# Autodesk Inventor assembly: Gripper Attempt 04
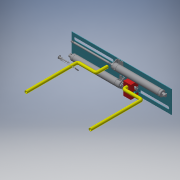
[picture p0: Inventor's stored thumbnail of the model, 180x180]
Saved by Autodesk Inventor 2016 (Build 200138000, 138)
## iProperties
Created: 2015-06-19
Part Number: Gripper Attempt 04
Document SubType Name: Assembly
Designer: steele
Mass: 1782.14 g
Surface Area: 5525.09 cm^2
Volume: 900.724 cm^3
Density: 1.97857 g/cm^3
Author: steele
## Documents named in this file (9)
- C:\snobotics\CAD-Development\robSteele\SnoBoticsSummer2015\Gripper\Gripper Attempt 04.iam
- C:\snobotics\CAD-MfgResources\McMaster-Carr\Air Cylinder\Pivot Mount Cylinders\Foot Bracket for 1_25 and 1_50 Bore\6498K340.ipt
- C:\snobotics\CAD-Development\robSteele\SnoBoticsSummer2015\Gripper\6498K681.ipt
- C:\snobotics\CAD-Development\robSteele\ipartComponents\Plate for Gripper.ipt
- C:\snobotics\CAD-Development\robSteele\ipartComponents\Plate for Gripper\Plate for Gripper 6 x 27 x 1_8.ipt
- C:\snobotics\CAD-Development\robSteele\SnoBoticsSummer2015\Gripper\Support For Arms.ipt
- C:\snobotics\CAD-Development\robSteele\SnoBoticsSummer2015\Gripper\Support Overlay on Gripper Side.ipt
- C:\snobotics\CAD-Development\robSteele\ipartComponents\ABS Arm.ipt
- C:\snobotics\CAD-MfgResources\McMaster-Carr\Quick Release Pin\94748A227.ipt
## Components (11 placed, 7 different names)
1. Plate for Gripper 6 x 27 x 1_8:1 — Mate:1, Flush:1, Flush:2, Mate:2, Flush:3, Flush:4, Mate:9
2. 6498K340:1 — Mate:2, Flush:3, Flush:4, Mate:7
3. 6498K340:2 — Mate:1, Flush:1, Flush:2, Mate:8
4. 6498K681:1 — Mate:7
5. 6498K681:2 — Mate:8, Insert:3
6. Support For Arms:1 — Mate:9, Insert:3, Mate:10, Flush:10, Flush:13, Mate:12
7. Support Overlay on Gripper Side:1 — Mate:10, Flush:10, Flush:13, Mate:12, Insert:4, Insert:5
8. ABS Arm:1 — Insert:4
9. ABS Arm:2
10. 94748A227:1 — Insert:5
11. 94748A227:2
## Relationships (16: Mate 7, Flush 6, Insert 3)
- Mate:1: Plate for Gripper 6 x 27 x 1_8:1 ↔ 6498K340:2
- Flush:1: Plate for Gripper 6 x 27 x 1_8:1 ↔ 6498K340:2
- Flush:2 (330.2 mm): Plate for Gripper 6 x 27 x 1_8:1 ↔ 6498K340:2
- Mate:2: Plate for Gripper 6 x 27 x 1_8:1 ↔ 6498K340:1
- Flush:3: Plate for Gripper 6 x 27 x 1_8:1 ↔ 6498K340:1
- Flush:4 (330.2 mm): Plate for Gripper 6 x 27 x 1_8:1 ↔ 6498K340:1
- Mate:7: 6498K340:1 ↔ 6498K681:1
- Mate:8: 6498K340:2 ↔ 6498K681:2
- Mate:9: Plate for Gripper 6 x 27 x 1_8:1 ↔ Support For Arms:1
- Insert:3: 6498K681:2 ↔ Support For Arms:1
- Mate:10: Support For Arms:1 ↔ Support Overlay on Gripper Side:1
- Flush:10: Support For Arms:1 ↔ Support Overlay on Gripper Side:1
- Flush:13: Support For Arms:1 ↔ Support Overlay on Gripper Side:1
- Mate:12: Support For Arms:1 ↔ Support Overlay on Gripper Side:1
- Insert:4 (-50.8 mm): Support Overlay on Gripper Side:1 ↔ ABS Arm:1
- Insert:5: Support Overlay on Gripper Side:1 ↔ 94748A227:1
## Named parameters: offsetToFrontOfAirCylinder = 330.2 mm
